# Autodesk Inventor assembly: 3U_generic_Mar1_4 Stack
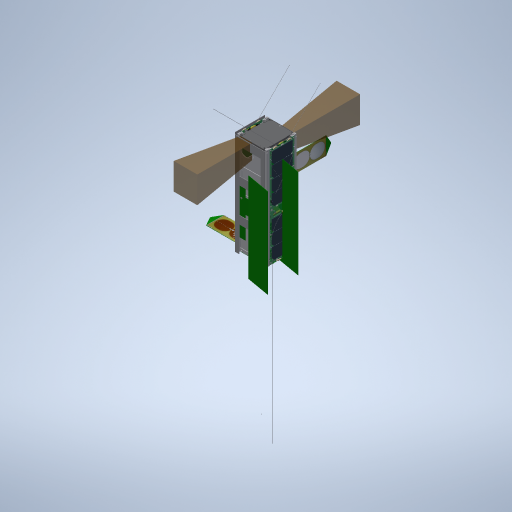
[picture p0: Inventor's stored thumbnail of the model, 512x512]
Saved by Autodesk Inventor 2023 (Build 270158000, 158)
## iProperties
Created: 2017-09-26
Part Number: 3U_generic_Mar1_4 Stack
Document SubType Name: Assembly
Designer: RDavis
Author: RDavis
## iProperties of the stored document MemberDocs/xAaaaajdaAaaaaaaaAaaaqnovDh
Created: 2017-09-26
Part Number: 3U_generic_Mar1_4 Stack
Document SubType Name: Assembly
Designer: RDavis
Author: RDavis
## Documents named in this file (20)
- E:\Dropbox\AMSAT\CAD_backup_frequent_files_20200629\Mar1\3U_generic_Mar1_4 Stack.iam
- E:\Dropbox\AMSAT\CAD_backup_frequent_files_20200629\3U_SP_generic_array.iam
- E:\Dropbox\AMSAT\CAD_backup_frequent_files_20200629\3U_sq_tube_amsat.iam
- E:\Dropbox\AMSAT\CAD_backup_frequent_files_20200629\3U_sq_tube_ragnorak.iam
- E:\Dropbox\AMSAT\CAD_backup_frequent_files_20200629\3U_SP_generic_rear.iam
- E:\Dropbox\AMSAT\CAD_backup_frequent_files_20200629\90318A201_ULP_SHLDR_SCREW_1-8_4-40.ipt
- E:\Dropbox\AMSAT\CAD_backup_frequent_files_20200629\P-POD_Access_Panels.ipt
- E:\Dropbox\AMSAT\CAD_backup_frequent_files_20200629\_-Z.iam
- E:\Dropbox\AMSAT\CAD_backup_frequent_files_20200629\Imported Components\90910A682_lpbhtorx_2-56_1-4\90910A682_lpbhtorx_2-56_1-4.ipt
- E:\Dropbox\AMSAT\CAD_backup_frequent_files_20200629\MS21043-04.ipt
- E:\Dropbox\AMSAT\CAD_backup_frequent_files_20200629\90945A713_NAS620C5_flat_washer.ipt
- E:\Dropbox\AMSAT\CAD_backup_frequent_files_20200629\90945A710_NAS620C4L_flat_washer.ipt
- E:\Dropbox\AMSAT\CAD_backup_frequent_files_20200629\Imported Components\92185A077_SHCS_2-56_1-4\92185A077_SHCS_2-56_1-4.ipt
- E:\Dropbox\AMSAT\CAD_backup_frequent_files_20200629\washer_nas620c2.ipt
- E:\Dropbox\AMSAT\CAD_backup_frequent_files_20200629\Imported Components\92196A075_SHCS_2-56_5-32\92196A075_SHCS_2-56_5-32.ipt
- E:\Dropbox\AMSAT\CAD_backup_frequent_files_20200629\Imported Components\90910A781_lpbhtorx_2-56_1-8\90910A781_lpbhtorx_2-56_1-8.ipt
- E:\Dropbox\AMSAT\CAD_backup_frequent_files_20200629\CSTT_wires_conn.iam
- E:\Dropbox\AMSAT\Cube Sat Frame Info\ISIS\ISIS CubeSat STS PC104 Skeleton-MAR1.iam
- E:\Dropbox\AMSAT\CAD_backup_frequent_files_20200629\nub_minusZ_1.ipt
- E:\Dropbox\AMSAT\CAD_backup_frequent_files_20200629\3U_generic.iam
## Components (51 placed, 16 different names)
1. 3U_sq_tube_ragnorak:3 [sub-assembly] — Insert:1, Insert:2, Flush:34, Flush:35, Mate:27, Flush:44, Flush:45, Flush:46, Insert:42, Insert:43, Insert:44, Insert:45, Insert:46, Insert:47
2. 3U_sq_tube_amsat:1 [sub-assembly] — Flush:34, Flush:35, Mate:27, Mate:28, Flush:36, Flush:37, Mate:29, Flush:38, Flush:39, Flush:41, Insert:6, Mate:33, Insert:8, Insert:15, Angle:1, Mate:50, Flush:6
3. 90318A201_ULP_SHLDR_SCREW_1-8_4-40:1 — Insert:1
4. 90318A201_ULP_SHLDR_SCREW_1-8_4-40:2 — Insert:2
5. 90318A201_ULP_SHLDR_SCREW_1-8_4-40:3 — Insert:42
6. 90318A201_ULP_SHLDR_SCREW_1-8_4-40:4 — Insert:43
7. 3U_SP_generic_array:1 [sub-assembly] — Flush:6, Mate:50
8. 3U_SP_generic_array:2 [sub-assembly] — Flush:8, Mate:33
9. 3U_SP_generic_rear:1 [sub-assembly] — Insert:15, Angle:1, Insert:16, Insert:17, Insert:18, Insert:19, Insert:20, Insert:21, Insert:22, Insert:23, Insert:24, Insert:25
10. washer_nas620c2:1 — Insert:16, Insert:26
11. washer_nas620c2:2 — Insert:17, Insert:30
12. washer_nas620c2:3 — Insert:18, Insert:31
13. washer_nas620c2:4 — Insert:19, Insert:32
14. washer_nas620c2:5 — Insert:20, Insert:28
15. washer_nas620c2:6 — Insert:21, Insert:27
16. washer_nas620c2:7 — Insert:22, Insert:33
17. washer_nas620c2:8 — Insert:23, Insert:34
18. washer_nas620c2:9 — Insert:24, Insert:35
19. washer_nas620c2:10 — Insert:25, Insert:29
20. 92185A077_SHCS_2-56_1-4:1 — Insert:26
21. 92185A077_SHCS_2-56_1-4:2 — Insert:27
22. 92185A077_SHCS_2-56_1-4:3 — Insert:28
23. 92185A077_SHCS_2-56_1-4:4 — Insert:29
24. 92196A075_SHCS_2-56_5-32:1 — Insert:30
25. 92196A075_SHCS_2-56_5-32:2 — Insert:31
26. 92196A075_SHCS_2-56_5-32:3 — Insert:32
27. 92196A075_SHCS_2-56_5-32:4 — Insert:33
28. 92196A075_SHCS_2-56_5-32:5 — Insert:34
29. 92196A075_SHCS_2-56_5-32:6 — Insert:35
30. P-POD_Access_Panels:1 — Mate:28, Flush:36, Flush:37
31. P-POD_Access_Panels:2 — Mate:29, Flush:38, Flush:39
32. _-Z:1 [sub-assembly] — Flush:41, Flush:42, Flush:43
33. 90945A713_NAS620C5_flat_washer:1 — Insert:6, Insert:7
34. 90945A710_NAS620C4L_flat_washer:1 — Insert:7, Insert:5
35. MS21043-04:1 — Insert:5
36. 3U_SP_generic_rear:2 [sub-assembly] — Flush:47, Insert:8, Insert:11, Insert:12, Insert:13, Insert:14, Insert:36, Insert:37, Insert:38, Insert:39, Insert:40, Insert:41
37. 90910A682_lpbhtorx_2-56_1-4:5 — Insert:11
38. 90910A682_lpbhtorx_2-56_1-4:6 — Insert:12
39. 90910A682_lpbhtorx_2-56_1-4:7 — Insert:13
40. 90910A682_lpbhtorx_2-56_1-4:8 — Insert:14
41. 90910A781_lpbhtorx_2-56_1-8:1 — Insert:36
42. 90910A781_lpbhtorx_2-56_1-8:2 — Insert:37
43. 90910A781_lpbhtorx_2-56_1-8:3 — Insert:38
44. 90910A781_lpbhtorx_2-56_1-8:4 — Insert:39
45. 90910A781_lpbhtorx_2-56_1-8:5 — Insert:40
46. 90910A781_lpbhtorx_2-56_1-8:6 — Insert:41
47. 90318A201_ULP_SHLDR_SCREW_1-8_4-40:5 — Insert:44
48. 90318A201_ULP_SHLDR_SCREW_1-8_4-40:6 — Insert:45
49. 90318A201_ULP_SHLDR_SCREW_1-8_4-40:7 — Insert:46
50. 90318A201_ULP_SHLDR_SCREW_1-8_4-40:8 — Insert:47
51. CSTT_wires_conn:1 [sub-assembly]
## Relationships (66: Insert 44, Flush 15, Mate 5, Angle 2)
- Flush:6 (9 mm): 3U_sq_tube_amsat:1 ↔ 3U_SP_generic_array:1
- Flush:8: 3U_SP_generic_array:2
- Insert:1: 3U_sq_tube_ragnorak:3 ↔ 90318A201_ULP_SHLDR_SCREW_1-8_4-40:1
- Insert:2: 3U_sq_tube_ragnorak:3 ↔ 90318A201_ULP_SHLDR_SCREW_1-8_4-40:2
- Flush:34: 3U_sq_tube_ragnorak:3 ↔ 3U_sq_tube_amsat:1
- Flush:35: 3U_sq_tube_ragnorak:3 ↔ 3U_sq_tube_amsat:1
- Mate:27: 3U_sq_tube_ragnorak:3 ↔ 3U_sq_tube_amsat:1
- Mate:28 (6.5 mm): 3U_sq_tube_amsat:1 ↔ P-POD_Access_Panels:1
- Flush:36: 3U_sq_tube_amsat:1 ↔ P-POD_Access_Panels:1
- Flush:37: 3U_sq_tube_amsat:1 ↔ P-POD_Access_Panels:1
- Mate:29 (6.5 mm): 3U_sq_tube_amsat:1 ↔ P-POD_Access_Panels:2
- Flush:38: 3U_sq_tube_amsat:1 ↔ P-POD_Access_Panels:2
- Flush:39: 3U_sq_tube_amsat:1 ↔ P-POD_Access_Panels:2
- Flush:41 (2 mm): 3U_sq_tube_amsat:1 ↔ _-Z:1
- Flush:42: _-Z:1
- Flush:43: _-Z:1
- Flush:44: 3U_sq_tube_ragnorak:3
- Flush:45: 3U_sq_tube_ragnorak:3
- Flush:46: 3U_sq_tube_ragnorak:3
- Insert:5: 90945A710_NAS620C4L_flat_washer:1 ↔ MS21043-04:1
- Insert:6: 3U_sq_tube_amsat:1 ↔ 90945A713_NAS620C5_flat_washer:1
- Insert:7: 90945A713_NAS620C5_flat_washer:1 ↔ 90945A710_NAS620C4L_flat_washer:1
- Mate:33: 3U_sq_tube_amsat:1 ↔ 3U_SP_generic_array:2
- Flush:47: 3U_SP_generic_rear:2
- Insert:8: 3U_sq_tube_amsat:1 ↔ 3U_SP_generic_rear:2
- Insert:11: 3U_SP_generic_rear:2 ↔ 90910A682_lpbhtorx_2-56_1-4:5
- Insert:12: 3U_SP_generic_rear:2 ↔ 90910A682_lpbhtorx_2-56_1-4:6
- Insert:13: 3U_SP_generic_rear:2 ↔ 90910A682_lpbhtorx_2-56_1-4:7
- Insert:14: 3U_SP_generic_rear:2 ↔ 90910A682_lpbhtorx_2-56_1-4:8
- Insert:15: 3U_sq_tube_amsat:1 ↔ 3U_SP_generic_rear:1
- Angle:1 (0 deg): 3U_sq_tube_amsat:1 ↔ 3U_SP_generic_rear:1
- Insert:16: 3U_SP_generic_rear:1 ↔ washer_nas620c2:1
- Insert:17: 3U_SP_generic_rear:1 ↔ washer_nas620c2:2
- Insert:18: 3U_SP_generic_rear:1 ↔ washer_nas620c2:3
- Insert:19: 3U_SP_generic_rear:1 ↔ washer_nas620c2:4
- Insert:20: 3U_SP_generic_rear:1 ↔ washer_nas620c2:5
- Insert:21: 3U_SP_generic_rear:1 ↔ washer_nas620c2:6
- Insert:22: 3U_SP_generic_rear:1 ↔ washer_nas620c2:7
- Insert:23: 3U_SP_generic_rear:1 ↔ washer_nas620c2:8
- Insert:24: 3U_SP_generic_rear:1 ↔ washer_nas620c2:9
- Insert:25: 3U_SP_generic_rear:1 ↔ washer_nas620c2:10
- Insert:26: washer_nas620c2:1 ↔ 92185A077_SHCS_2-56_1-4:1
- Insert:27: washer_nas620c2:6 ↔ 92185A077_SHCS_2-56_1-4:2
- Insert:28: washer_nas620c2:5 ↔ 92185A077_SHCS_2-56_1-4:3
- Insert:29: washer_nas620c2:10 ↔ 92185A077_SHCS_2-56_1-4:4
- Insert:30: washer_nas620c2:2 ↔ 92196A075_SHCS_2-56_5-32:1
- Insert:31: washer_nas620c2:3 ↔ 92196A075_SHCS_2-56_5-32:2
- Insert:32: washer_nas620c2:4 ↔ 92196A075_SHCS_2-56_5-32:3
- Insert:33: washer_nas620c2:7 ↔ 92196A075_SHCS_2-56_5-32:4
- Insert:34: washer_nas620c2:8 ↔ 92196A075_SHCS_2-56_5-32:5
- Insert:35: washer_nas620c2:9 ↔ 92196A075_SHCS_2-56_5-32:6
- Insert:36: 3U_SP_generic_rear:2 ↔ 90910A781_lpbhtorx_2-56_1-8:1
- Insert:37: 3U_SP_generic_rear:2 ↔ 90910A781_lpbhtorx_2-56_1-8:2
- Insert:38: 3U_SP_generic_rear:2 ↔ 90910A781_lpbhtorx_2-56_1-8:3
- Insert:39: 3U_SP_generic_rear:2 ↔ 90910A781_lpbhtorx_2-56_1-8:4
- Insert:40: 3U_SP_generic_rear:2 ↔ 90910A781_lpbhtorx_2-56_1-8:5
- Insert:41: 3U_SP_generic_rear:2 ↔ 90910A781_lpbhtorx_2-56_1-8:6
- Insert:42: 3U_sq_tube_ragnorak:3 ↔ 90318A201_ULP_SHLDR_SCREW_1-8_4-40:3
- Insert:43: 3U_sq_tube_ragnorak:3 ↔ 90318A201_ULP_SHLDR_SCREW_1-8_4-40:4
- Insert:44: 3U_sq_tube_ragnorak:3 ↔ 90318A201_ULP_SHLDR_SCREW_1-8_4-40:5
- Insert:45: 3U_sq_tube_ragnorak:3 ↔ 90318A201_ULP_SHLDR_SCREW_1-8_4-40:6
- Insert:46: 3U_sq_tube_ragnorak:3 ↔ 90318A201_ULP_SHLDR_SCREW_1-8_4-40:7
- Insert:47: 3U_sq_tube_ragnorak:3 ↔ 90318A201_ULP_SHLDR_SCREW_1-8_4-40:8
- [Insert] (0.102 mm): 3U_sq_tube_ragnorak:3 ↔ CSTT_wires_conn:1
- [Angle] (0 deg): 3U_sq_tube_ragnorak:3 ↔ CSTT_wires_conn:1
- Mate:50: 3U_sq_tube_amsat:1 ↔ 3U_SP_generic_array:1
## Named parameters: deploy = 45 deg
